# Autodesk Inventor assembly: fly_funnel_combinations
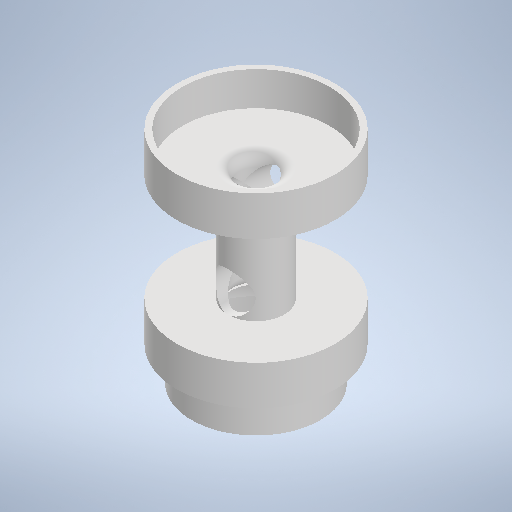
[picture p0: Inventor's stored thumbnail of the model, 512x512]
Saved by Autodesk Inventor 2025 (Build 290162010, 162A)
## iProperties
Created: 2023-05-01
Part Number: fly_funnel_combinations
Document SubType Name: Assembly
Designer: dinesh
Author: dinesh
## Documents named in this file (3)
- C:\Users\dinesh\Documents\GitHub\flytools\flyporter\fly_funnel_combinations.iam
- C:\Users\dinesh\Documents\GitHub\flytools\flyporter\vial\archive\vial_adapter_female.ipt
- C:\Users\dinesh\Documents\GitHub\flytools\flyporter\vial\archive\vial_adapter_male.ipt
## Components (2 placed, 2 different names)
1. vial_adapter_female:1 — Mate:1, Mate:2
2. vial_adapter_male:1 — Mate:1, Mate:2
## Relationships (2: Mate 2)
- Mate:1: vial_adapter_female:1 ↔ vial_adapter_male:1
- Mate:2: vial_adapter_female:1 ↔ vial_adapter_male:1
